# Autodesk Inventor assembly: Pen Holder Assembly V2
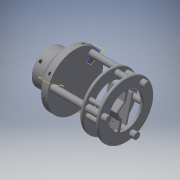
[picture p0: Inventor's stored thumbnail of the model, 180x180]
Saved by Autodesk Inventor 2019 (Build 230136000, 136)
## iProperties
Created: 2019-07-22
Part Number: Pen Holder Assembly V2
Document SubType Name: Assembly
Designer: Matthew XPS
Author: Matthew XPS
## Documents named in this file (6)
- G:\My Drive\Documents\Human Robot Interaction Lab\Projects\2019-06 Adept Viper Robot Arm\Pen  Holder\Pen Holder Assembly V2.iam
- G:\My Drive\Documents\Human Robot Interaction Lab\Projects\2019-06 Adept Viper Robot Arm\Pen  Holder\Pen Interface V2.ipt
- G:\My Drive\Documents\Human Robot Interaction Lab\Projects\2019-06 Adept Viper Robot Arm\Pen  Holder\10mm Rod.ipt
- G:\My Drive\Documents\Human Robot Interaction Lab\Projects\2019-06 Adept Viper Robot Arm\Pen  Holder\Spring 2mm for 10mm rod.ipt
- G:\My Drive\Documents\Human Robot Interaction Lab\Projects\2019-06 Adept Viper Robot Arm\Pen  Holder\Pen Main Piece V3.ipt
- G:\My Drive\Documents\Human Robot Interaction Lab\Projects\2019-06 Adept Viper Robot Arm\Pen  Holder\Clamp Plate V2.ipt
## Components (7 placed, 5 different names)
1. Pen Interface V2:1 — Rigid:1, Rigid:2, Rigid:3
2. 10mm Rod:1 — Rigid:1, Mate:1
3. 10mm Rod:2 — Rigid:2
4. 10mm Rod:3 — Rigid:3, Mate:3
5. Spring 2mm for 10mm rod:1
6. Pen Main Piece V3:1 — Mate:1, Mate:2, Mate:3, Angle:1
7. Clamp Plate V2:1 — Mate:2, Angle:1
## Relationships (7: WeldJoint 3, Mate 3, Angle 1)
- Rigid:1 [WeldJoint]: Pen Interface V2:1 ↔ 10mm Rod:1
- Rigid:2 [WeldJoint]: Pen Interface V2:1 ↔ 10mm Rod:2
- Rigid:3 [WeldJoint]: Pen Interface V2:1 ↔ 10mm Rod:3
- Mate:1: 10mm Rod:1 ↔ Pen Main Piece V3:1
- Mate:2: Pen Main Piece V3:1 ↔ Clamp Plate V2:1
- Mate:3: 10mm Rod:3 ↔ Pen Main Piece V3:1
- Angle:1 (0 deg): Pen Main Piece V3:1 ↔ Clamp Plate V2:1
